# Autodesk Inventor assembly: motorEaro
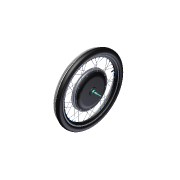
[picture p0: Inventor's stored thumbnail of the model, 180x180]
Saved by Autodesk Inventor 2015 (Build 190159000, 159)
## iProperties
Created: 2016-08-29
Part Number: motorEaro
Document SubType Name: Assembly
Designer: EriveltonDell
Author: EriveltonDell
## Documents named in this file (3)
- C:\Users\EriveltonDell\Documents\Centro Universitário da FEI\Power-Assisted-Wheelchair-master\Power-Assisted-Wheelchair-master\motorEaro.iam
- C:\Users\EriveltonDell\Documents\Centro Universitário da FEI\Power-Assisted-Wheelchair-master\Power-Assisted-Wheelchair-master\Importowane komponenty\Hub_Motor_MagicPie2_ASM\Hub_Motor_MagicPie2_ASM.iam
- C:\Users\EriveltonDell\Documents\Centro Universitário da FEI\Power-Assisted-Wheelchair-master\Power-Assisted-Wheelchair-master\Ciąg.iam
## Components (2 placed, 2 different names)
1. Hub_Motor_MagicPie2_ASM:1 [sub-assembly]
2. Ciąg:1 [sub-assembly]
## Relationships (1: Mate 1)
- [Mate]: Hub_Motor_MagicPie2_ASM:1 ↔ Ciąg:1
